# Autodesk Inventor assembly: 4 Traction, Circle_MIR
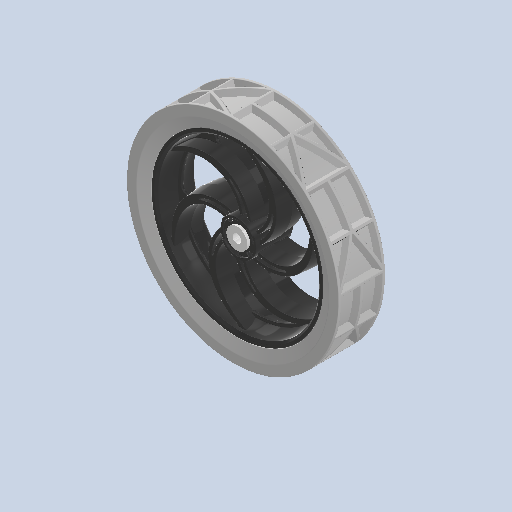
[picture p0: Inventor's stored thumbnail of the model, 512x512]
Saved by Autodesk Inventor 2024 (Build 280153000, 153)
## iProperties
Created: 2022-08-02
Part Number: 4 Traction, Circle_MIR
Document SubType Name: Assembly
Designer: ismae
Author: ylu12
## Documents named in this file (3)
- C:\Users\ismae\Desktop\VEX\CAD 2023\VEX-CAD-Inventor\Motion\Wheels\Traction Wheel\4 Traction, Circle_MIR.iam
- C:\Users\ismae\Desktop\VEX\CAD 2023\VEX-CAD-Inventor\Motion\Wheels\Reference Files\4 Traction_MIR.ipt
- C:\Users\ismae\Desktop\VEX\CAD 2023\VEX-CAD-Inventor\Motion\Insert Circle_MIR1.ipt
## Components (3 placed, 2 different names)
1. 4 Traction_MIR:1 — Coincidencia:12, Coincidencia:11, Nivelación:6
2. Insert Circle_MIR1:1 — Ángulo:4, Coincidencia:29, Simetría:2
3. Insert Circle_MIR1:2 — Simetría:2, Ángulo:3, Coincidencia:26, Nivelación:11
## Relationships (9: Mate 5, Angle 2, Flush 1, Symmetry 1)
- Coincidencia:12 [Mate]: 4 Traction_MIR:1
- Coincidencia:11 [Mate]: 4 Traction_MIR:1
- Nivelación:6 [Flush]: 4 Traction_MIR:1
- Ángulo:4 [Angle] (0 deg): Insert Circle_MIR1:1
- Coincidencia:29 [Mate]: Insert Circle_MIR1:1
- Simetría:2 [Symmetry]: Insert Circle_MIR1:1 ↔ Insert Circle_MIR1:2
- Ángulo:3 [Angle] (0 deg): Insert Circle_MIR1:2
- Coincidencia:26 [Mate]: Insert Circle_MIR1:2
- Nivelación:11 [Mate] (8.255 mm): Insert Circle_MIR1:2
## Named parameters: Thickness = 8.255 mm
